# Autodesk Inventor assembly: hand_fin1_opp
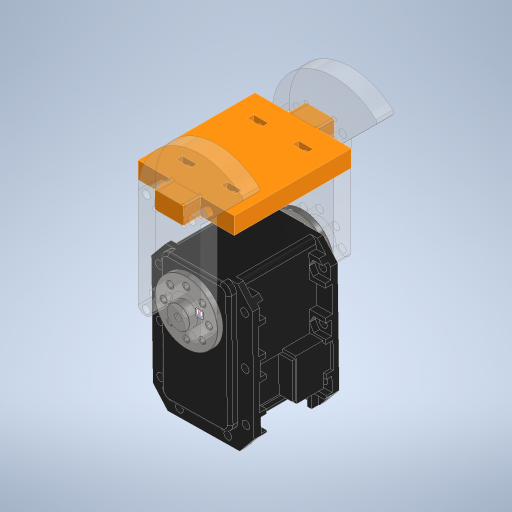
[picture p0: Inventor's stored thumbnail of the model, 512x512]
Saved by Autodesk Inventor 2024 (Build 280153000, 153)
## iProperties
Created: 2024-09-15
Part Number: hand_fin1_opp
Document SubType Name: Assembly
Designer: jmha0
Author: jmha0
## Documents named in this file (6)
- C:\Users\jmha0\OneDrive\바탕 화면\19th_intern_hjm_fight_robot\Upper_Body\hand\hand_fin1_opp.iam
- C:\Users\jmha0\OneDrive\바탕 화면\19th_intern_hjm_fight_robot\hardware\ROBOTIS(Inventor 2024 ver.)\다이나믹셀\MX-28T_R+idle.ipt.iam
- C:\Users\jmha0\OneDrive\바탕 화면\19th_intern_hjm_fight_robot\hardware\ROBOTIS(Inventor 2024 ver.)\혼\28Horn.ipt
- C:\Users\jmha0\OneDrive\바탕 화면\19th_intern_hjm_fight_robot\Upper_Body\hand\frame_hand1.ipt
- C:\Users\jmha0\OneDrive\바탕 화면\19th_intern_hjm_fight_robot\Upper_Body\hand\bridge_hands1.ipt
- MX-28T_R+idle.ipt
## Components (5 placed, 4 different names)
1. MX-28T_R+idle.ipt:1 [sub-assembly] — 삽입:10
2. 28Horn:1 — 삽입:11, 삽입:12
3. frame_hand1:1 — 삽입:11, 삽입:12
4. frame_hand1:2 — 삽입:10
5. bridge_hands1:1
## Relationships (6: Insert 6)
- [Insert] (0.1 mm): MX-28T_R+idle.ipt:1 ↔ 28Horn:1
- [Insert]: frame_hand1:2 ↔ bridge_hands1:1
- [Insert]: frame_hand1:1 ↔ bridge_hands1:1
- 삽입:10 [Insert]: MX-28T_R+idle.ipt:1 ↔ frame_hand1:2
- 삽입:11 [Insert]: 28Horn:1 ↔ frame_hand1:1
- 삽입:12 [Insert]: 28Horn:1 ↔ frame_hand1:1
## Named parameters: d3_d7 = 0 mm, d4_d8 = 0 mm
